# Autodesk Inventor assembly: Assembly_Raspberrypi
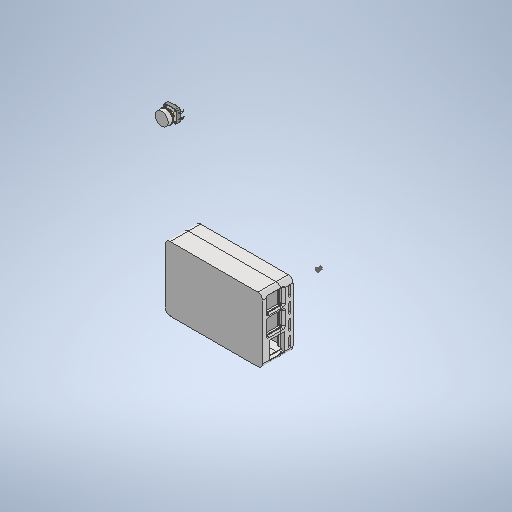
[picture p0: Inventor's stored thumbnail of the model, 512x512]
Saved by Autodesk Inventor 2025.2 (Build 292293000, 293)
## iProperties
Created: 2026-02-21
Part Number: Assembly_Raspberrypi
Document SubType Name: Assembly
Designer: naka6
Author: naka6
## iProperties of the stored document OMRON B3F 12mm TACT SWITCH.ipt
Created: 2021-10-02
Part Number: OMRON B3F 12mm TACT SWITCH
Material: 一般
Description: STEP AP214
Document SubType Name: Modeling
Designer: naka6
Density: 1 g/cm^3
Appearance: 既定
Title: OMRON B3F 12mm TACT SWITCH.STEP
Author: Alexrolex
Revision Number: ANY
Sending System: SolidWorks 2020
Preprocessor: SwSTEP 2.0
## Documents named in this file (8)
- **C:\Users\naka6\Projects\TimeFaker\Assembly_Raspberrypi.iam*LocalDocs*xAaaaqncaAaaaaaaaAaaaaigj2e*OMRON B3F 12mm TACT SWITCH.ipt
- C:\Users\naka6\Projects\TimeFaker\Assembly_Raspberrypi.iam
- C:\Users\naka6\Projects\TimeFaker\rohs-step-motor-28byj-48-1.snapshot.5\Step - 28BYJ-48\on switch.ipt
- C:\Users\naka6\Projects\TimeFaker\Cap.ipt
- C:\Users\naka6\Projects\TimeFaker\Part6.ipt
- C:\Users\naka6\Projects\TimeFaker\Part7.ipt
- C:\Users\naka6\Projects\TimeFaker\Part8.ipt
- C:\Users\naka6\Projects\TimeFaker\omron-b3f-12mm-tact-switch-1.snapshot.1\omron B3F\OMRON B3F 12mm TACT SWITCH.STEP
## Components (6 placed, 6 different names)
1. on switch:1
2. OMRON B3F 12mm TACT SWITCH:1
3. Cap:1
4. Part6:1 — フラッシュ:2, メイト:1, フラッシュ:3
5. Part7:1
6. Part8:1 — フラッシュ:2, メイト:1, フラッシュ:3
## Relationships (3: Flush 2, Mate 1)
- フラッシュ:2 [Flush]: Part6:1 ↔ Part8:1
- メイト:1 [Mate]: Part6:1 ↔ Part8:1
- フラッシュ:3 [Flush]: Part6:1 ↔ Part8:1
